# Autodesk Inventor assembly: fgdfgdfgd
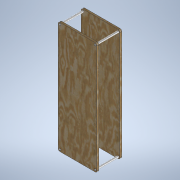
[picture p0: Inventor's stored thumbnail of the model, 180x180]
Saved by Autodesk Inventor 2020.2 (Build 242310000, 310)
## iProperties
Created: 2020-08-20
Part Number: fgdfgdfgd
Document SubType Name: Assembly
Designer: JK
Author: JK
## Documents named in this file (3)
- C:\Users\JK\Documents\Inventor\Anet Upgrade\fgdfgdfgd.iam
- C:\Users\JK\Documents\Inventor\Anet Upgrade\Tabletop.ipt
- C:\Users\JK\Documents\Inventor\Anet Upgrade\Altube.ipt
## Components (6 placed, 2 different names)
1. Tabletop:1 — Mate:1, Mate:2, Mate:3, Mate:4, Flush:1, Flush:2, Flush:3, Flush:4, Flush:6
2. Tabletop:2 — Mate:5, Flush:5, Flush:6
3. Altube:1 — Mate:1, Flush:4
4. Altube:2 — Mate:4, Flush:1
5. Altube:3 — Mate:3, Flush:2
6. Altube:4 — Mate:2, Flush:3, Mate:5, Flush:5
## Relationships (11: Flush 6, Mate 5)
- Mate:1: Tabletop:1 ↔ Altube:1
- Mate:2: Tabletop:1 ↔ Altube:4
- Mate:3: Tabletop:1 ↔ Altube:3
- Mate:4: Tabletop:1 ↔ Altube:2
- Flush:1: Tabletop:1 ↔ Altube:2
- Flush:2: Tabletop:1 ↔ Altube:3
- Flush:3: Tabletop:1 ↔ Altube:4
- Flush:4: Tabletop:1 ↔ Altube:1
- Mate:5: Tabletop:2 ↔ Altube:4
- Flush:5: Tabletop:2 ↔ Altube:4
- Flush:6: Tabletop:1 ↔ Tabletop:2
